# Autodesk Inventor assembly: Water Collection Sytem
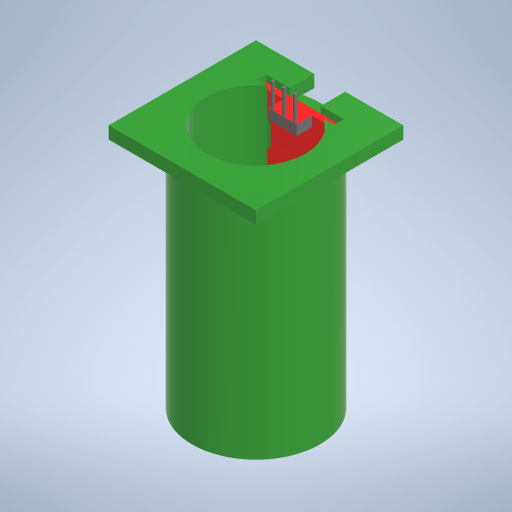
[picture p0: Inventor's stored thumbnail of the model, 512x512]
Saved by Autodesk Inventor 2023 (Build 270158000, 158)
## iProperties
Created: 2023-09-26
Part Number: Water Collection Sytem
Document SubType Name: Assembly
Designer: Gage
Author: Gage
## Documents named in this file (3)
- C:\Users\Gage\OneDrive\Desktop\Autodesk Inventor\207\Water Collection Sytem.iam
- C:\Users\Gage\OneDrive\Desktop\Autodesk Inventor\207\Water Sensor.ipt
- C:\Users\Gage\OneDrive\Desktop\Autodesk Inventor\207\WaterBucket2.ipt
## Components (2 placed, 2 different names)
1. Water Sensor:1 — Mate:1, Mate:2, Mate:3
2. WaterBucket2:1 — Mate:1, Mate:2, Mate:3
## Relationships (3: Mate 3)
- Mate:1: Water Sensor:1 ↔ WaterBucket2:1
- Mate:2: Water Sensor:1 ↔ WaterBucket2:1
- Mate:3: Water Sensor:1 ↔ WaterBucket2:1
